# Autodesk Inventor assembly: Thermal Camera Cover Assembly
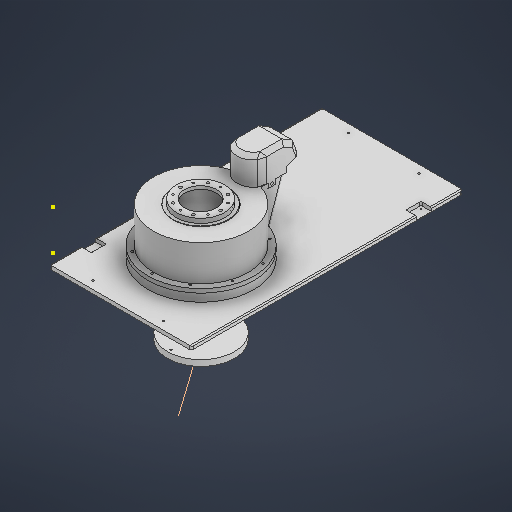
[picture p0: Inventor's stored thumbnail of the model, 512x512]
Saved by Autodesk Inventor 2026.1 (Build 301233000, 233)
## iProperties
Created: 2025-08-06
Part Number: Thermal Camera Cover Assembly
Document SubType Name: Assembly
Designer: mayhe
Author: mayhe
## Documents named in this file (11)
- C:\GitHub\In-situ-monitoring-of-powder-bed-fusion-additive-manufacturing\system_development\Adamant\v0.2\hardware_development\Thermal Camera Cover Assembly.iam
- C:\GitHub\In-situ-monitoring-of-powder-bed-fusion-additive-manufacturing\system_development\Adamant\v0.2\hardware_development\Cover parts\12mm Cover.ipt
- C:\GitHub\In-situ-monitoring-of-powder-bed-fusion-additive-manufacturing\system_development\Adamant\v0.2\hardware_development\Cover parts\SealedGlassRing.ipt
- C:\GitHub\In-situ-monitoring-of-powder-bed-fusion-additive-manufacturing\system_development\Adamant\v0.2\hardware_development\Cover parts\Xi-410-Camera-with-29°-x-18°-Lens\Xi 410 Camera with 29° x.iam
- C:\GitHub\In-situ-monitoring-of-powder-bed-fusion-additive-manufacturing\system_development\Adamant\v0.2\hardware_development\Cover parts\substrate plate.ipt
- C:\GitHub\In-situ-monitoring-of-powder-bed-fusion-additive-manufacturing\system_development\Adamant\v0.2\hardware_development\Cover parts\Cylinder Segment Holder.ipt
- C:\GitHub\In-situ-monitoring-of-powder-bed-fusion-additive-manufacturing\system_development\Adamant\v0.2\hardware_development\Cover parts\C .Replace - Face.ipt
- C:\GitHub\In-situ-monitoring-of-powder-bed-fusion-additive-manufacturing\system_development\Adamant\v0.2\hardware_development\Cover parts\Cylinder Segment Camera Only.ipt
- C:\GitHub\In-situ-monitoring-of-powder-bed-fusion-additive-manufacturing\system_development\Adamant\v0.2\hardware_development\Cover parts\Cylinder Segment Camera Only\C .Replace - 10.ipt
- C:\GitHub\In-situ-monitoring-of-powder-bed-fusion-additive-manufacturing\system_development\Adamant\v0.2\hardware_development\Cover parts\Cylinder Housing Camera v0.2.11.0015.ipt
- C:\GitHub\In-situ-monitoring-of-powder-bed-fusion-additive-manufacturing\system_development\Adamant\v0.2\hardware_development\Cover parts\lid - Copy.0011.ipt
## Components (9 placed, 9 different names)
1. 12mm Cover:1 — Rotational:1, Mate:1, Rotational:4
2. SealedGlassRing:1 — Rotational:1, Mate:1, Rotational:5
3. Xi 410 Camera with 29° x:1 [sub-assembly]
4. substrate plate:1 — Rotational:4
5. Cylinder Segment Holder:1 — Mate:3
6. C .Replace - Face:1 — Insert:2
7. C .Replace - 10:2 — Mate:3, Insert:2
8. Cylinder Housing Camera v0.2.11.0015:1 — Rotational:5, Mate:4, Rotational:6
9. lid - Copy.0011:1 — Mate:4, Rotational:6
## Relationships (8: RevoluteJoint 4, Mate 3, Insert 1)
- Rotational:1 [RevoluteJoint]: 12mm Cover:1 ↔ SealedGlassRing:1
- Mate:1: 12mm Cover:1 ↔ SealedGlassRing:1
- Rotational:4 [RevoluteJoint] (-150 mm): 12mm Cover:1 ↔ substrate plate:1
- Mate:3: Cylinder Segment Holder:1 ↔ C .Replace - 10:2
- Insert:2 (-15 mm): C .Replace - Face:1 ↔ C .Replace - 10:2
- Rotational:5 [RevoluteJoint]: SealedGlassRing:1 ↔ Cylinder Housing Camera v0.2.11.0015:1
- Mate:4: Cylinder Housing Camera v0.2.11.0015:1 ↔ lid - Copy.0011:1
- Rotational:6 [RevoluteJoint]: Cylinder Housing Camera v0.2.11.0015:1 ↔ lid - Copy.0011:1
